# Autodesk Inventor assembly: 1376426 DSBC-32-100-PPVA-N3---(0)
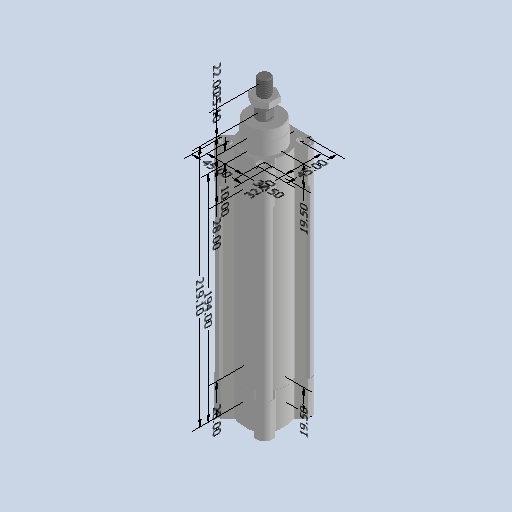
[picture p0: Inventor's stored thumbnail of the model, 512x512]
Saved by Autodesk Inventor 2025.1 (Build 291241000, 241)
## iProperties
Created: 2025-06-06
Part Number: 1376426 DSBC-32-100-PPVA-N3---(0)
Catalog Web Link: www.cadenas.de
Description: DSBC-Standard cylinder
Vendor: FESTO
Document SubType Name: Assembly
Designer: psAdmin
Manufacturer: FESTO
Mass: 735 g
Surface Area: 851.401 cm^2
Volume: 237.766 cm^3
Density: 3.09128 g/cm^3
Category: PARTsolutions
Company: FESTO
PSOL_IDENT_0: {ATYP=ASSISTANT},{DATA=script=$CADENAS_DATA/23d-libs/festo/webfesto.vbb&M_FAMILY=DSBC&M_GROUP=01&M_P
PSOL_IDENT_1: ARTNO=1376426&IDCODE1=DSBC-32-100-PPVA-N3&IDCODE2=&customer_number_cns=&MATES=1&LOD=HI&LOCKERP=0&SIN
PSOL_IDENT_2: GLEPART=1}
NB: 1376426 DSBC-32-100-PPVA-N3---(0)
NN: DSBC
NT: Standard cylinder
NBSYN: $TNR. $TYP.-$KDM.-$HUB.$PRFAT.-$DAE.A-$NOR.---($HUBST.)
LINA: 1376426 DSBC-32-100-PPVA-N3
CATALOG: Festo
OFFICIAL_STANDARD_NUMBERS: ISO 15552
TNR: 1376426
TYP: DSBC
KDM: 32
HUB: 100
HUBST: 0
PRFA: -
DAE: PPV
NOR: N3
A: 22
AM: 22
AF: 12
B: 30
BG: 16
E: 45
EB: 0
EE: G1/8
G: 28
U1: 5.25
U2: 5.7
KK: M10x1.25
L2: 18
L3: 4
L7: 6.5
L8: 194
MM: 12
PL: 19.5
RT: M6
TG: 32.5
VA: 4
VD: 10
WH: 25
ZJ: 219.1
SW1: 10
SW2: 16
SW3: 6
D1: 6.4
KF: M6
T1: 16
T2: 2.6
CNSMASSEXACT: 0.735
GTIN: 4052568016586
REACH: Yes
REACHSVHC: No
REACHHAZSUBS: -
REACHSCIP: -
REACHVALDATE: -
SUPPLIER: FESTO
ARTICLENO: 1376426 DSBC-32-100-PPVA-N3---(0)
BOMINFO: 1376426 DSBC-32-100-PPVA-N3
CREATOR: CADENAS GmbH
Title: 1376426 DSBC-32-100-PPVA-N3
Author: Cadenas PARTsolutions
Comments: Standard cylinder
## Documents named in this file (4)
- C:\Users\Erik\Erik\Hochschule\3. Semester\CAD\CAD-Paspa\Useless Box\Kaufteile\Festo_Normzylinder_100\1376426 DSBC-32-100-PPVA-N3---(0).iam
- C:\Users\Erik\Erik\Hochschule\3. Semester\CAD\CAD-Paspa\Useless Box\Kaufteile\Festo_Normzylinder_100\1463250 DSBC-32-100-PPVA_(Z_0).ipt
- C:\Users\Erik\Erik\Hochschule\3. Semester\CAD\CAD-Paspa\Useless Box\Kaufteile\Festo_Normzylinder_100\1463250 DSBC-32-100_(K).ipt
- C:\Users\Erik\Erik\Hochschule\3. Semester\CAD\CAD-Paspa\Useless Box\Kaufteile\Festo_Normzylinder_100\DIN-439-B - M10x1_25(F).ipt
## Components (3 placed, 3 different names)
1. 1463250 DSBC-32-100-PPVA_(Z_0):1 — 2P_XY@1 <-> P_XY@2, 2P_Z@1 <-> P_Z@2, 2P_YZ@1 <-> P_YZ@2
2. 1463250 DSBC-32-100_(K):1 — 2P_XY@1 <-> P_XY@2, 2P_Z@1 <-> P_Z@2, 2P_YZ@1 <-> P_YZ@2, NUT_XY@2 <-> din439b_punkt_XY@3, NUT_Z@2 <-> din439b_punkt_Z@3, NUT_YZ@2 <-> din439b_punkt_YZ@3
3. DIN-439-B - M10x1_25(F):1 — NUT_XY@2 <-> din439b_punkt_XY@3, NUT_Z@2 <-> din439b_punkt_Z@3, NUT_YZ@2 <-> din439b_punkt_YZ@3
## Relationships (6: Mate 4, Angle 2)
- 2P_XY@1 <-> P_XY@2 [Mate]: 1463250 DSBC-32-100-PPVA_(Z_0):1 ↔ 1463250 DSBC-32-100_(K):1
- 2P_Z@1 <-> P_Z@2 [Mate]: 1463250 DSBC-32-100-PPVA_(Z_0):1 ↔ 1463250 DSBC-32-100_(K):1
- 2P_YZ@1 <-> P_YZ@2 [Angle] (90 deg): 1463250 DSBC-32-100-PPVA_(Z_0):1 ↔ 1463250 DSBC-32-100_(K):1
- NUT_XY@2 <-> din439b_punkt_XY@3 [Mate]: 1463250 DSBC-32-100_(K):1 ↔ DIN-439-B - M10x1_25(F):1
- NUT_Z@2 <-> din439b_punkt_Z@3 [Mate]: 1463250 DSBC-32-100_(K):1 ↔ DIN-439-B - M10x1_25(F):1
- NUT_YZ@2 <-> din439b_punkt_YZ@3 [Angle] (0 deg): 1463250 DSBC-32-100_(K):1 ↔ DIN-439-B - M10x1_25(F):1
